# Autodesk Inventor assembly: Remote Assembly
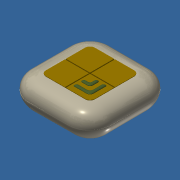
[picture p0: Inventor's stored thumbnail of the model, 180x180]
Saved by Autodesk Inventor 2016 (Build 200138000, 138)
## iProperties
Created: 2015-06-16
Part Number: Remote Assembly
Document SubType Name: Assembly
Designer: Samuel Clay
Author: Samuel Clay
## Documents named in this file (8)
- Z:\enclosure\inventor\Remote Assembly.iam
- Z:\enclosure\inventor\Remote Top.ipt
- Z:\enclosure\inventor\Remote Bottom.ipt
- Z:\enclosure\inventor\Remote Buttons.ipt
- Z:\enclosure\inventor\Eagle PCB rev 21.ipt
- Z:\enclosure\inventor\Case Bottom.ipt
- Z:\enclosure\inventor\Case Top.ipt
- Z:\enclosure\inventor\Case Buttons.ipt
## Components (7 placed, 7 different names)
1. Remote Top:1 — Mate:1, Mate:9, Mate:10
2. Remote Buttons:1 — Mate:1, Mate:2, Mate:6, Mate:8, Mate:11
3. Remote Bottom:1 — Rotational:1
4. Case Top:1 — Mate:5, Mate:6, Mate:10, Mate:12
5. Case Bottom:1 — Mate:5, Mate:9, Mate:12
6. Case Buttons:1 — Mate:2, Mate:8, Mate:11
7. Eagle PCB rev 21:1 — Rotational:1
## Relationships (10: Mate 9, RevoluteJoint 1)
- Mate:1: Remote Top:1 ↔ Remote Buttons:1
- Mate:2: Remote Buttons:1 ↔ Case Buttons:1
- Rotational:1 [RevoluteJoint]: Remote Bottom:1 ↔ Eagle PCB rev 21:1
- Mate:5: Case Top:1 ↔ Case Bottom:1
- Mate:6: Remote Buttons:1 ↔ Case Top:1
- Mate:8: Remote Buttons:1 ↔ Case Buttons:1
- Mate:9: Remote Top:1 ↔ Case Bottom:1
- Mate:10: Remote Top:1 ↔ Case Top:1
- Mate:11: Remote Buttons:1 ↔ Case Buttons:1
- Mate:12: Case Top:1 ↔ Case Bottom:1
